# Autodesk Inventor assembly: MountedScanners
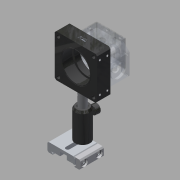
[picture p0: Inventor's stored thumbnail of the model, 180x180]
Saved by Autodesk Inventor 2018 (Build 220112000, 112)
## iProperties
Created: 2018-09-24
Part Number: MountedScanners
Document SubType Name: Assembly
Designer: Robert Campbell
Author: Robert Campbell
## Documents named in this file (6)
- X:\home\work\Documents\MF_BenchOptics\CAD_files\MountedScanners.iam
- W:\home\work\Documents\MF_BenchOptics\CAD_files\GCM102_M-Solidworks.ipt
- W:\home\work\Documents\MF_BenchOptics\CAD_files\LCP11_M-Solidworks.ipt
- W:\home\work\Documents\MF_BenchOptics\CAD_files\PH50_M-Solidworks.ipt
- W:\home\work\Documents\MF_BenchOptics\CAD_files\TR50_M-Solidworks.ipt
- W:\home\work\Documents\MF_BenchOptics\CAD_files\XT66C4-Step.ipt
## Components (5 placed, 5 different names)
1. GCM102_M-Solidworks:1 — Mate:1, Mate:2, Angle:1
2. LCP11_M-Solidworks:1 — Mate:1, Mate:2, Angle:1, Mate:7, Mate:8, Angle:2
3. PH50_M-Solidworks:1 — Mate:3, Mate:4, Mate:5, Mate:6
4. TR50_M-Solidworks:1 — Mate:3, Mate:4, Mate:7, Mate:8
5. XT66C4-Step:1 — Mate:5, Mate:6, Angle:2
## Relationships (10: Mate 8, Angle 2)
- Mate:1: GCM102_M-Solidworks:1 ↔ LCP11_M-Solidworks:1
- Mate:2: GCM102_M-Solidworks:1 ↔ LCP11_M-Solidworks:1
- Angle:1 (0 deg): GCM102_M-Solidworks:1 ↔ LCP11_M-Solidworks:1
- Mate:3: PH50_M-Solidworks:1 ↔ TR50_M-Solidworks:1
- Mate:4 (20 mm): PH50_M-Solidworks:1 ↔ TR50_M-Solidworks:1
- Mate:5: PH50_M-Solidworks:1 ↔ XT66C4-Step:1
- Mate:6: PH50_M-Solidworks:1 ↔ XT66C4-Step:1
- Mate:7: LCP11_M-Solidworks:1 ↔ TR50_M-Solidworks:1
- Mate:8: LCP11_M-Solidworks:1 ↔ TR50_M-Solidworks:1
- Angle:2 (0 deg): LCP11_M-Solidworks:1 ↔ XT66C4-Step:1
